# Autodesk Inventor assembly: Right Angle Structure
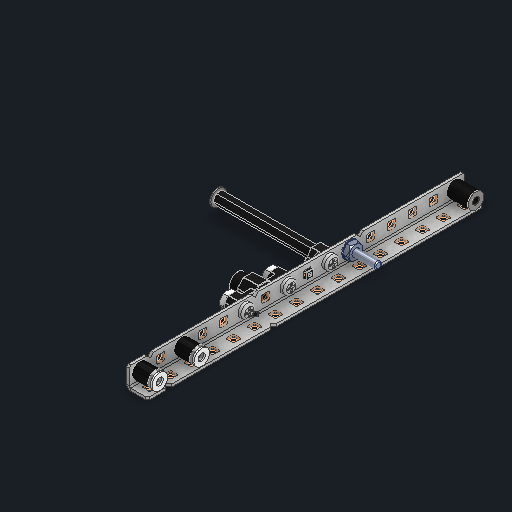
[picture p0: Inventor's stored thumbnail of the model, 512x512]
Saved by Autodesk Inventor 2025.1 (Build 291241000, 241)
## iProperties
Created: 2024-10-20
Part Number: Right Angle Structure
Document SubType Name: Assembly
Designer: Averey Ku
Author: Averey Ku
## Documents named in this file (24)
- C:\Users\avere\VEX\High Stakes\CAD\V3\Intake\Right Angle Structure\Right Angle Structure.iam
- C:\Users\avere\VEX\High Stakes\CAD\V3\Intake\Right Angle Structure\Right Alu Angle 1x1x16.ipt
- C:\Users\avere\VEX\High Stakes\CAD\ROBOPROS-CAD-Inventor\Motion\Spacers\Spacer Nylon .375 OD\NSpacer .375 OD x .500.ipt
- C:\Users\avere\VEX\High Stakes\CAD\ROBOPROS-CAD-Inventor\Motion\Spacers\Washer Steel\SWasher .375 OD x .015625.ipt
- C:\Users\avere\VEX\High Stakes\CAD\V3\Intake\Right Angle Structure\Right HS Bearing Flat.ipt
- C:\Users\avere\VEX\High Stakes\CAD\ROBOPROS-CAD-Inventor\Structure\Hardware\Nut Nylon\Nut Nylon - White.ipt
- C:\Users\avere\VEX\High Stakes\CAD\ROBOPROS-CAD-Inventor\Motion\Spacers\Spacer Nylon .375 OD\NSpacer .375 OD x .375.ipt
- C:\Users\avere\VEX\High Stakes\CAD\ROBOPROS-CAD-Inventor\Motion\Spacers\Washer Steel\SWasher .375 OD x .062500.ipt
- C:\Users\avere\VEX\High Stakes\CAD\ROBOPROS-CAD-Inventor\Motion\Spacers\Washer Teflon\TWasher .375 OD x .04000.ipt
- C:\Users\avere\VEX\High Stakes\CAD\ROBOPROS-CAD-Inventor\Motion\Spacers\Spacer Nylon .375 OD.ipt
- C:\Users\avere\VEX\High Stakes\CAD\ROBOPROS-CAD-Inventor\Motion\Spacers\Washer Steel.ipt
- C:\Users\avere\VEX\High Stakes\CAD\ROBOPROS-CAD-Inventor\Structure\Hardware\Nut Nylon.ipt
- C:\Users\avere\VEX\High Stakes\CAD\ROBOPROS-CAD-Inventor\Motion\Spacers\Washer Teflon.ipt
- C:\Users\avere\VEX\High Stakes\CAD\ROBOPROS-CAD-Inventor\Structure\1-Post Standoff Retainer.ipt
- C:\Users\avere\VEX\High Stakes\CAD\ROBOPROS-CAD-Inventor\Structure\Standoff\Standoff 2.50.ipt
- C:\Users\avere\VEX\High Stakes\CAD\ROBOPROS-CAD-Inventor\Structure\Standoff.ipt
- C:\Users\avere\VEX\High Stakes\CAD\ROBOPROS-CAD-Inventor\Structure\Hardware\Screw Nylon - Pan Head\NScrew Pan Head Threaded .375.ipt
- C:\Users\avere\VEX\High Stakes\CAD\ROBOPROS-CAD-Inventor\Motion\Spacers\Washer Steel\SWasher .375 OD x .031250.ipt
- C:\Users\avere\VEX\High Stakes\CAD\ROBOPROS-CAD-Inventor\Motion\Shaft HS\HS Spacer\HSpacer .2500.ipt
- C:\Users\avere\VEX\High Stakes\CAD\ROBOPROS-CAD-Inventor\Motion\Shaft HS\HS Spacer.ipt
- C:\Users\avere\VEX\High Stakes\CAD\ROBOPROS-CAD-Inventor\Structure\Hardware\Screw Nylon - Pan Head\NScrew Pan Head Threaded .500.ipt
- C:\Users\avere\VEX\High Stakes\CAD\ROBOPROS-CAD-Inventor\Structure\Hardware\Screw Steel - Star\SScrew Star Smooth .750.ipt
- C:\Users\avere\VEX\High Stakes\CAD\ROBOPROS-CAD-Inventor\Structure\Hardware\Screw Steel - Star.ipt
- C:\Users\avere\VEX\High Stakes\CAD\ROBOPROS-CAD-Inventor\Structure\Hardware\Nut Keps.ipt
## Components (21 placed, 16 different names)
1. Right Alu Angle 1x1x16:1 — Mate:2, Mate:1, Flush:1, Insert:3, Mate:4, Insert:4, Insert:11, Insert:14, Insert:19, Mate:7, Insert:21, Insert:22, Insert:23, Insert:24
2. NSpacer .375 OD x .500:1 — Insert:3, Insert:2
3. SWasher .375 OD x .015625:1 — Insert:2
4. Right HS Bearing Flat:1 — Mate:4, Insert:4, Insert:5, Insert:6
5. Nut Nylon - White:1 — Insert:5
6. Nut Nylon - White:2 — Insert:6
7. NSpacer .375 OD x .375:2 — Insert:11, Insert:10
8. SWasher .375 OD x .062500:2 — Insert:10, Insert:9
9. TWasher .375 OD x .04000:1 — Insert:9
10. NSpacer .375 OD x .375:3 — Insert:14, Insert:13
11. SWasher .375 OD x .062500:3 — Insert:13, Insert:12
12. TWasher .375 OD x .04000:2 — Insert:12
13. 1-Post Standoff Retainer:1 — Mate:7
14. Standoff 2.50:1
15. NScrew Pan Head Threaded .375:1 — Insert:19
16. SWasher .375 OD x .031250:4
17. HSpacer .2500:1
18. NScrew Pan Head Threaded .500:1 — Insert:22
19. NScrew Pan Head Threaded .500:2 — Insert:21
20. SScrew Star Smooth .750:1 — Insert:23
21. Nut Keps:1 — Insert:24
## Relationships (25: Insert 19, Mate 5, Angle 1)
- Mate:2: Right Alu Angle 1x1x16:1
- Mate:1: Right Alu Angle 1x1x16:1
- Flush:1 [Mate] (-101.6 mm): Right Alu Angle 1x1x16:1
- Insert:3: Right Alu Angle 1x1x16:1 ↔ NSpacer .375 OD x .500:1
- Insert:2: NSpacer .375 OD x .500:1 ↔ SWasher .375 OD x .015625:1
- Mate:4: Right Alu Angle 1x1x16:1 ↔ Right HS Bearing Flat:1
- Insert:4: Right Alu Angle 1x1x16:1 ↔ Right HS Bearing Flat:1
- Insert:5: Right HS Bearing Flat:1 ↔ Nut Nylon - White:1
- Insert:6: Right HS Bearing Flat:1 ↔ Nut Nylon - White:2
- Insert:11: Right Alu Angle 1x1x16:1 ↔ NSpacer .375 OD x .375:2
- Insert:10: NSpacer .375 OD x .375:2 ↔ SWasher .375 OD x .062500:2
- Insert:9: SWasher .375 OD x .062500:2 ↔ TWasher .375 OD x .04000:1
- Insert:14: Right Alu Angle 1x1x16:1 ↔ NSpacer .375 OD x .375:3
- Insert:13: NSpacer .375 OD x .375:3 ↔ SWasher .375 OD x .062500:3
- Insert:12: SWasher .375 OD x .062500:3 ↔ TWasher .375 OD x .04000:2
- [Insert]: 1-Post Standoff Retainer:1 ↔ Standoff 2.50:1
- [Angle] (0 deg): 1-Post Standoff Retainer:1 ↔ Standoff 2.50:1
- [Insert] (1.5875 mm): 1-Post Standoff Retainer:1 ↔ NScrew Pan Head Threaded .375:1
- [Insert]: Standoff 2.50:1 ↔ SWasher .375 OD x .031250:4
- Insert:19: Right Alu Angle 1x1x16:1 ↔ NScrew Pan Head Threaded .375:1
- Mate:7: Right Alu Angle 1x1x16:1 ↔ 1-Post Standoff Retainer:1
- Insert:21: Right Alu Angle 1x1x16:1 ↔ NScrew Pan Head Threaded .500:2
- Insert:22: Right Alu Angle 1x1x16:1 ↔ NScrew Pan Head Threaded .500:1
- Insert:23: Right Alu Angle 1x1x16:1 ↔ SScrew Star Smooth .750:1
- Insert:24: Right Alu Angle 1x1x16:1 ↔ Nut Keps:1
